# Autodesk Inventor assembly: Wheel 75 mm Assembly
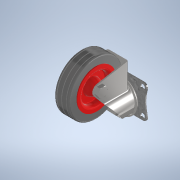
[picture p0: Inventor's stored thumbnail of the model, 180x180]
Saved by Autodesk Inventor 2020 (Build 240168000, 168)
## iProperties
Created: 2023-01-26
Part Number: Wheel 75 mm Assembly
Document SubType Name: Assembly
Designer: saad.nashed
Author: saad.nashed
## Documents named in this file (13)
- D:\Wheel diameter 75 mm\Wheel 75 mm Assembly.iam
- D:\E\Air Cooler Start in 2022\Air Cooler\Common Files\Wheels\Wheel 75 mm - Part 1.ipt
- D:\E\Air Cooler Start in 2022\Air Cooler\Common Files\Wheels\Wheel 75 mm - Part 3.ipt
- D:\Wheel diameter 75 mm\Wheel 75 mm - Part 1.ipt
- D:\Wheel diameter 75 mm\Wheel 75 mm - Part 2.ipt
- D:\Wheel diameter 75 mm\Wheel 75 mm - Part 3.ipt
- D:\Wheel diameter 75 mm\DIN 960 - M8 x 1 x 40.ipt
- D:\Wheel diameter 75 mm\DIN 934 - M8 x 1.25.ipt
- D:\Wheel diameter 75 mm\AS 1968 - 1976 - 8.ipt
- D:\Wheel diameter 75 mm\Wheel 75 mm - Part 4.ipt
- D:\Wheel diameter 75 mm\Wheel 75 mm - Part 5.ipt
- D:\Wheel diameter 75 mm\Wheel 75 mm - Part 6.ipt
- D:\Wheel diameter 75 mm\Ball.ipt
## Components (21 placed, 10 different names)
1. Wheel 75 mm - Part 1:3 — Mate:1, Tangent:3, Mate:3, Mate:5, Mate:6, Mate:21
2. Wheel 75 mm - Part 2:1 — Mate:3, Mate:5, Mate:7, Mate:21
3. Wheel 75 mm - Part 3:3 — Mate:6, Mate:7, Mate:8, Mate:9, Mate:10, Mate:14, Mate:15, Mate:22, Mate:16, Mate:17, Mate:18
4. DIN 960 - replaced by DIN EN 28765 M8 x 1 x 40:1 — Mate:8, Mate:9, Mate:11, Mate:12
5. DIN 934 - replaced by DIN EN 24032/28673/28674 M8:1 — Mate:11, Mate:13
6. AS 1968 8:1 — Mate:10, Mate:12, Mate:13
7. Wheel 75 mm - Part 4:1 — Mate:14, Mate:16, Mate:23
8. Wheel 75 mm - Part 5:1 — Mate:17, Mate:18, Mate:19
9. Wheel 75 mm - Part 6:1 — Mate:19, Mate:23, Mate:20
10. Ball:13 — Mate:15, Mate:22
11. Ball:14
12. Ball:15
13. Ball:16
14. Ball:17
15. Ball:18
16. Ball:19
17. Ball:20
18. Ball:21
19. Ball:22
20. Ball:23
21. Ball:24
## Component patterns: (12 elements, first: Ball:13)
## Relationships (22: Mate 21, Tangent 1)
- Mate:1: Wheel 75 mm - Part 1:3
- Tangent:3: Wheel 75 mm - Part 1:3
- Mate:3: Wheel 75 mm - Part 1:3 ↔ Wheel 75 mm - Part 2:1
- Mate:5: Wheel 75 mm - Part 1:3 ↔ Wheel 75 mm - Part 2:1
- Mate:6: Wheel 75 mm - Part 1:3 ↔ Wheel 75 mm - Part 3:3
- Mate:7: Wheel 75 mm - Part 2:1 ↔ Wheel 75 mm - Part 3:3
- Mate:8: Wheel 75 mm - Part 3:3 ↔ DIN 960 - replaced by DIN EN 28765 M8 x 1 x 40:1
- Mate:9: Wheel 75 mm - Part 3:3 ↔ DIN 960 - replaced by DIN EN 28765 M8 x 1 x 40:1
- Mate:10: Wheel 75 mm - Part 3:3 ↔ AS 1968 8:1
- Mate:11: DIN 960 - replaced by DIN EN 28765 M8 x 1 x 40:1 ↔ DIN 934 - replaced by DIN EN 24032/28673/28674 M8:1
- Mate:12: DIN 960 - replaced by DIN EN 28765 M8 x 1 x 40:1 ↔ AS 1968 8:1
- Mate:13: DIN 934 - replaced by DIN EN 24032/28673/28674 M8:1 ↔ AS 1968 8:1
- Mate:14: Wheel 75 mm - Part 3:3 ↔ Wheel 75 mm - Part 4:1
- Mate:15 (13.1769 mm): Wheel 75 mm - Part 3:3 ↔ Ball:13
- Mate:22 (-3.8625 mm): Wheel 75 mm - Part 3:3 ↔ Ball:13
- Mate:16 (1.5 mm): Wheel 75 mm - Part 3:3 ↔ Wheel 75 mm - Part 4:1
- Mate:17: Wheel 75 mm - Part 3:3 ↔ Wheel 75 mm - Part 5:1
- Mate:18: Wheel 75 mm - Part 3:3 ↔ Wheel 75 mm - Part 5:1
- Mate:19: Wheel 75 mm - Part 5:1 ↔ Wheel 75 mm - Part 6:1
- Mate:23: Wheel 75 mm - Part 4:1 ↔ Wheel 75 mm - Part 6:1
- Mate:20: Wheel 75 mm - Part 6:1
- Mate:21: Wheel 75 mm - Part 1:3 ↔ Wheel 75 mm - Part 2:1
## Named parameters: d0_1 = 37.5 mm
